# Autodesk Inventor assembly: WheelAssembly
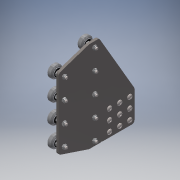
[picture p0: Inventor's stored thumbnail of the model, 180x180]
Saved by Autodesk Inventor 2017 (Build 210142000, 142)
## iProperties
Created: 2016-12-12
Part Number: WheelAssembly
Document SubType Name: Assembly
Designer: umr
Mass: 4376.08 g
Surface Area: 10170.9 cm^2
Volume: 1553.17 cm^3
Density: 2.81752 g/cm^3
Author: umr
## Documents named in this file (4)
- D:\SeniorProject\Models2\WheelAssembly\WheelAssembly.iam
- D:\SeniorProject\Models2\Gantry\Gantry Plate.ipt
- D:\SeniorProject\Models2\Gantry\M5 Screw with Tee Nut.iam
- D:\SeniorProject\Models2\Gantry\Solid Wheel with Eccentric Spacer Assembly.iam
## Components (19 placed, 3 different names)
1. Solid Wheel with Eccentric Spacer Assembly:2 [sub-assembly] — Mate:26, Mate:40
2. Gantry Plate:1 — Mate:1, Mate:2, Mate:3, Mate:4, Mate:5, Mate:6, Mate:7, Mate:8, Mate:9, Mate:11, Mate:12, Mate:13, Mate:14, Mate:16, Mate:17, Mate:18, Mate:21, Mate:22, Mate:26, Mate:27, Mate:28, Mate:29, Mate:30, Mate:31, Mate:32, Mate:33, Mate:34, Mate:35, Mate:36, Mate:37, Mate:38, Mate:39, Mate:40, Mate:41, Mate:42, Mate:43
3. Solid Wheel with Eccentric Spacer Assembly:5 [sub-assembly] — Mate:30, Mate:42
4. Solid Wheel with Eccentric Spacer Assembly:1 [sub-assembly] — Mate:29, Mate:43
5. Solid Wheel with Eccentric Spacer Assembly:4 [sub-assembly] — Mate:28, Mate:41
6. Solid Wheel with Eccentric Spacer Assembly:3 [sub-assembly] — Mate:27, Mate:39
7. Solid Wheel with Eccentric Spacer Assembly:6 [sub-assembly] — Mate:31, Mate:35
8. Solid Wheel with Eccentric Spacer Assembly:7 [sub-assembly] — Mate:32, Mate:36
9. Solid Wheel with Eccentric Spacer Assembly:8 [sub-assembly] — Mate:33, Mate:37
10. Solid Wheel with Eccentric Spacer Assembly:10 [sub-assembly] — Mate:34, Mate:38
11. M5 Screw with Tee Nut:4 [sub-assembly] — Mate:5, Mate:18
12. M5 Screw with Tee Nut:8 [sub-assembly] — Mate:9, Mate:17
13. M5 Screw with Tee Nut:1 [sub-assembly] — Mate:1, Mate:2
14. M5 Screw with Tee Nut:3 [sub-assembly] — Mate:4, Mate:11
15. M5 Screw with Tee Nut:2 [sub-assembly] — Mate:3, Mate:14
16. M5 Screw with Tee Nut:7 [sub-assembly] — Mate:8, Mate:16
17. M5 Screw with Tee Nut:9 [sub-assembly] — Mate:21, Mate:22
18. M5 Screw with Tee Nut:6 [sub-assembly] — Mate:7, Mate:13
19. M5 Screw with Tee Nut:5 [sub-assembly] — Mate:6, Mate:12
## Relationships (36: Mate 36)
- Mate:1: Gantry Plate:1 ↔ M5 Screw with Tee Nut:1
- Mate:2: Gantry Plate:1 ↔ M5 Screw with Tee Nut:1
- Mate:3: Gantry Plate:1 ↔ M5 Screw with Tee Nut:2
- Mate:4: Gantry Plate:1 ↔ M5 Screw with Tee Nut:3
- Mate:5: Gantry Plate:1 ↔ M5 Screw with Tee Nut:4
- Mate:6: Gantry Plate:1 ↔ M5 Screw with Tee Nut:5
- Mate:7: Gantry Plate:1 ↔ M5 Screw with Tee Nut:6
- Mate:8: Gantry Plate:1 ↔ M5 Screw with Tee Nut:7
- Mate:9: Gantry Plate:1 ↔ M5 Screw with Tee Nut:8
- Mate:11: Gantry Plate:1 ↔ M5 Screw with Tee Nut:3
- Mate:12: Gantry Plate:1 ↔ M5 Screw with Tee Nut:5
- Mate:13: Gantry Plate:1 ↔ M5 Screw with Tee Nut:6
- Mate:14: Gantry Plate:1 ↔ M5 Screw with Tee Nut:2
- Mate:16: Gantry Plate:1 ↔ M5 Screw with Tee Nut:7
- Mate:17: Gantry Plate:1 ↔ M5 Screw with Tee Nut:8
- Mate:18: Gantry Plate:1 ↔ M5 Screw with Tee Nut:4
- Mate:21: Gantry Plate:1 ↔ M5 Screw with Tee Nut:9
- Mate:22: Gantry Plate:1 ↔ M5 Screw with Tee Nut:9
- Mate:26: Solid Wheel with Eccentric Spacer Assembly:2 ↔ Gantry Plate:1
- Mate:27: Gantry Plate:1 ↔ Solid Wheel with Eccentric Spacer Assembly:3
- Mate:28: Gantry Plate:1 ↔ Solid Wheel with Eccentric Spacer Assembly:4
- Mate:29: Gantry Plate:1 ↔ Solid Wheel with Eccentric Spacer Assembly:1
- Mate:30: Gantry Plate:1 ↔ Solid Wheel with Eccentric Spacer Assembly:5
- Mate:31: Gantry Plate:1 ↔ Solid Wheel with Eccentric Spacer Assembly:6
- Mate:32: Gantry Plate:1 ↔ Solid Wheel with Eccentric Spacer Assembly:7
- Mate:33: Gantry Plate:1 ↔ Solid Wheel with Eccentric Spacer Assembly:8
- Mate:34: Gantry Plate:1 ↔ Solid Wheel with Eccentric Spacer Assembly:10
- Mate:35: Gantry Plate:1 ↔ Solid Wheel with Eccentric Spacer Assembly:6
- Mate:36: Gantry Plate:1 ↔ Solid Wheel with Eccentric Spacer Assembly:7
- Mate:37: Gantry Plate:1 ↔ Solid Wheel with Eccentric Spacer Assembly:8
- Mate:38: Gantry Plate:1 ↔ Solid Wheel with Eccentric Spacer Assembly:10
- Mate:39: Gantry Plate:1 ↔ Solid Wheel with Eccentric Spacer Assembly:3
- Mate:40: Solid Wheel with Eccentric Spacer Assembly:2 ↔ Gantry Plate:1
- Mate:41: Gantry Plate:1 ↔ Solid Wheel with Eccentric Spacer Assembly:4
- Mate:42: Gantry Plate:1 ↔ Solid Wheel with Eccentric Spacer Assembly:5
- Mate:43: Gantry Plate:1 ↔ Solid Wheel with Eccentric Spacer Assembly:1
